# Autodesk Inventor assembly: forkMountForDecTripV02
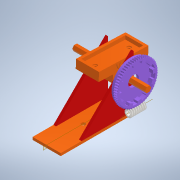
[picture p0: Inventor's stored thumbnail of the model, 180x180]
Saved by Autodesk Inventor 2021.2 (Build 252289000, 289)
## iProperties
Created: 2020-11-09
Part Number: forkMountForDecTripV02
Document SubType Name: Assembly
Designer: robst
Author: robst
## Documents named in this file (7)
- C:\git\CAD-Development\robSteele\ShapeWays\TelescopeProjects\TelescopeMount\forkMountForDecTripV02.iam
- C:\git\CAD-Development\robSteele\ShapeWays\TelescopeProjects\TelescopeMount\tripod.ipt
- C:\git\CAD-Development\robSteele\ShapeWays\TelescopeProjects\TelescopeMount\triangleSupportForMount.ipt
- C:\git\CAD-Development\robSteele\ShapeWays\TelescopeProjects\TelescopeMount\triangleBase.ipt
- C:\git\CAD-Development\robSteele\ShapeWays\TelescopeProjects\TelescopeMount\connectorToTubeBracketWithOffsetHexShaft-V01.ipt
- C:\git\CAD-Development\robSteele\ShapeWays\TelescopeProjects\TelescopeMount\hexBearing.ipt
- C:\git\CAD-Development\robSteele\ShapeWays\TelescopeProjects\TelescopeMount\forkMountForDecTripV01\Design Accelerator\Worm Gears5.iam
## Components (7 placed, 6 different names)
1. tripod:1 — Insert:1, Flush:5
2. triangleSupportForMount:1 — Mate:1, Flush:1, Flush:2, Insert:2
3. triangleBase:1 — Mate:1, Flush:1, Flush:2, Insert:1, Mate:2, Flush:3, Flush:4, Flush:5
4. triangleSupportForMount:2 — Mate:2, Flush:3, Flush:4
5. connectorToTubeBracketWithOffsetHexShaft-V01:1 — Mate:3, Mate:4, Mate:5
6. hexBearing:1 — Mate:3, Mate:4, Mate:5, Insert:2, Insert:3
7. Worm Gears:1 [sub-assembly] — Insert:3
## Relationships (13: Mate 5, Flush 5, Insert 3)
- Mate:1: triangleSupportForMount:1 ↔ triangleBase:1
- Flush:1: triangleSupportForMount:1 ↔ triangleBase:1
- Flush:2: triangleSupportForMount:1 ↔ triangleBase:1
- Insert:1: tripod:1 ↔ triangleBase:1
- Mate:2: triangleBase:1 ↔ triangleSupportForMount:2
- Flush:3: triangleBase:1 ↔ triangleSupportForMount:2
- Flush:4: triangleBase:1 ↔ triangleSupportForMount:2
- Mate:3: connectorToTubeBracketWithOffsetHexShaft-V01:1 ↔ hexBearing:1
- Mate:4: connectorToTubeBracketWithOffsetHexShaft-V01:1 ↔ hexBearing:1
- Mate:5: connectorToTubeBracketWithOffsetHexShaft-V01:1 ↔ hexBearing:1
- Insert:2: triangleSupportForMount:1 ↔ hexBearing:1
- Flush:5: tripod:1 ↔ triangleBase:1
- Insert:3 (12.7 mm): hexBearing:1 ↔ Worm Gears:1
